# Autodesk Inventor assembly: X-Motor-Housing
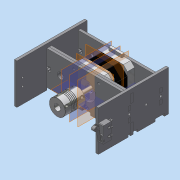
[picture p0: Inventor's stored thumbnail of the model, 180x180]
Saved by Autodesk Inventor 2016 SP1 (Build 200210100, 210)
## iProperties
Created: 2016-02-17
Part Number: X-Motor-Housing
Document SubType Name: Assembly
Designer: Mohamed A.
Mass: 241.707 g
Surface Area: 875.015 cm^2
Volume: 137.241 cm^3
Density: 1.76118 g/cm^3
Author: Mohamed A.
## Documents named in this file (7)
- C:\Users\Mohamed\Documents\inventor\StemCellsPlatform\Laser Cut\X-Motor Housing\X-Motor-Housing.iam
- C:\Users\Mohamed\Documents\inventor\StemCellsPlatform\Motors\NEMA-7-17HD34008-22B.ipt
- C:\Users\Mohamed\Documents\inventor\StemCellsPlatform\Laser Cut\X-Motor Housing\X-Motor-Housing_Front-Inner.ipt
- C:\Users\Mohamed\Documents\inventor\StemCellsPlatform\Laser Cut\X-Motor Housing\X-Motor-Housing_Front-Outer.ipt
- C:\Users\Mohamed\Documents\inventor\StemCellsPlatform\Laser Cut\X-Motor Housing\X-Motor-Housing_Side.ipt
- C:\Users\Mohamed\Documents\inventor\StemCellsPlatform\Couplers\Flexible Shaft CouplerAcople FlexibleSLDPRT.ipt
- C:\Users\Mohamed\Documents\inventor\StemCellsPlatform\Buttons\SPDT Limit Switch\605634.ipt
## Components (8 placed, 6 different names)
1. NEMA-7-17HD34008-22B:1 — Flush:1, Mate:1, Mate:2, Mate:3, Flush:2, Mate:4, Cylindrical:1, Flush:8, Mate:19
2. X-Motor-Housing_Front-Inner:1 — Flush:1, Mate:1, Mate:2, Flush:5, Flush:18, Mate:15, Mate:16, Flush:19, Mate:17, Mate:18, Flush:23
3. X-Motor-Housing_Front-Outer:1 — Flush:6, Mate:15, Mate:16, Flush:23
4. X-Motor-Housing_Front-Outer:2 — Flush:18, Flush:24, Mate:19
5. X-Motor-Housing_Side:1 — Flush:5, Flush:6, Mate:6, Mate:7, Mate:8
6. Flexible Shaft CouplerAcople FlexibleSLDPRT:1 — Cylindrical:1, Flush:8, Flush:9
7. 605634:1 — Mate:6, Flush:9, Mate:7, Mate:8
8. X-Motor-Housing_Side:2 — Flush:19, Mate:17, Mate:18, Flush:24
## Relationships (23: Mate 12, Flush 10, CylindricalJoint 1)
- Flush:1: NEMA-7-17HD34008-22B:1 ↔ X-Motor-Housing_Front-Inner:1
- Mate:1: NEMA-7-17HD34008-22B:1 ↔ X-Motor-Housing_Front-Inner:1
- Mate:2: NEMA-7-17HD34008-22B:1 ↔ X-Motor-Housing_Front-Inner:1
- Mate:3: NEMA-7-17HD34008-22B:1
- Flush:2: NEMA-7-17HD34008-22B:1
- Mate:4: NEMA-7-17HD34008-22B:1
- Flush:5: X-Motor-Housing_Front-Inner:1 ↔ X-Motor-Housing_Side:1
- Flush:6: X-Motor-Housing_Front-Outer:1 ↔ X-Motor-Housing_Side:1
- Cylindrical:1: NEMA-7-17HD34008-22B:1 ↔ Flexible Shaft CouplerAcople FlexibleSLDPRT:1
- Flush:8: NEMA-7-17HD34008-22B:1 ↔ Flexible Shaft CouplerAcople FlexibleSLDPRT:1
- Mate:6: X-Motor-Housing_Side:1 ↔ 605634:1
- Flush:9: Flexible Shaft CouplerAcople FlexibleSLDPRT:1 ↔ 605634:1
- Mate:7: X-Motor-Housing_Side:1 ↔ 605634:1
- Mate:8: X-Motor-Housing_Side:1 ↔ 605634:1
- Flush:18: X-Motor-Housing_Front-Inner:1 ↔ X-Motor-Housing_Front-Outer:2
- Mate:15: X-Motor-Housing_Front-Inner:1 ↔ X-Motor-Housing_Front-Outer:1
- Mate:16: X-Motor-Housing_Front-Inner:1 ↔ X-Motor-Housing_Front-Outer:1
- Flush:19: X-Motor-Housing_Front-Inner:1 ↔ X-Motor-Housing_Side:2
- Mate:17: X-Motor-Housing_Front-Inner:1 ↔ X-Motor-Housing_Side:2
- Mate:18: X-Motor-Housing_Front-Inner:1 ↔ X-Motor-Housing_Side:2
- Flush:23: X-Motor-Housing_Front-Inner:1 ↔ X-Motor-Housing_Front-Outer:1
- Flush:24: X-Motor-Housing_Front-Outer:2 ↔ X-Motor-Housing_Side:2
- Mate:19: NEMA-7-17HD34008-22B:1 ↔ X-Motor-Housing_Front-Outer:2
